# Autodesk Inventor assembly: Тиски
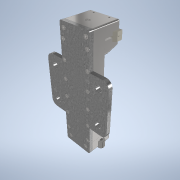
[picture p0: Inventor's stored thumbnail of the model, 180x180]
Saved by Autodesk Inventor 2020 (Build 240168000, 168)
## iProperties
Created: 2020-12-05
Part Number: Тиски
Document SubType Name: Assembly
Designer: User
Author: User
## Documents named in this file (18)
- F:\Детали\Тиски\Тиски.iam
- F:\Детали\Тиски\Основание.ipt
- F:\Детали\Тиски\Тиски\Мастер проектирования\Болтовое соединение1.iam
- F:\Детали\Тиски\Упор 1.ipt
- F:\Детали\Тиски\Упор 2.ipt
- F:\Детали\Тиски\Направляющая.ipt
- F:\Детали\Тиски\Тиски\Мастер проектирования\Болтовое соединение3.iam
- F:\Детали\Тиски\Губка.ipt
- F:\Детали\Тиски\Тиски\Мастер проектирования\Болтовое соединение5.iam
- F:\Детали\Тиски\Каретка.ipt
- F:\Детали\Тиски\Тиски\Мастер проектирования\Подшипник1.iam
- F:\Детали\Тиски\Вал1.ipt
- F:\Детали\Тиски\Фланец.ipt
- C:\Users\User\Documents\Inventor\Content Center Files\R2020\ru-RU\DIN 916\DIN 916 - M4  x  10.ipt
- F:\Детали\Тиски\Тиски\Мастер проектирования\Болтовое соединение7.iam
- F:\Детали\Тиски\Привод.iam
- F:\Детали\Тиски\Тиски\Мастер проектирования\Болтовое соединение8.iam
- F:\Детали\Тиски\Ручка.ipt
## Components (21 placed, 13 different names)
1. Основание:1 — Заподлицо:1, Совмещение:4, Совмещение:5, Совмещение:6, Совмещение:7, Совмещение:8, Совмещение:9, Совмещение:10, Совмещение:11, Совмещение:12, Совмещение:13, Совмещение:14, Совмещение:15, Совмещение:17, Совмещение:19, Совмещение:21, Совмещение:23, Совмещение:25, Совмещение:27, Совмещение:29, Совмещение:31, Совмещение:33, Совмещение:35, Совмещение:40, Совмещение:41, Совмещение:42, Совмещение:43, Совмещение:44, Совмещение:46, Совмещение:48, Совмещение:50, Совмещение:57, Совмещение:59, Совмещение:61, Жесткий:1, Жесткий:2, Жесткий:3, Совмещение:82, Совмещение:83, Совмещение:93
2. Болтовое соединение:1 [sub-assembly] — Совмещение:59, Совмещение:60, Совмещение:61
3. Упор 1:1 — Жесткий:2, Жесткий:4, С поворотом:2
4. Упор 2:1 — Жесткий:3, С поворотом:1
5. Направляющая:1 — Жесткий:1, Совмещение:81, Угол:1
6. Болтовое соединение:2 [sub-assembly] — Совмещение:93, Совмещение:94
7. Губка:1 — Жесткий:4, Совмещение:70, Совмещение:71, Совмещение:72, Совмещение:74, Совмещение:76
8. Болтовое соединение:3 [sub-assembly] — Совмещение:76, Совмещение:77
9. Каретка:1 — Совмещение:80, Совмещение:81, ЗубчПер:1, Жесткий:8
10. Подшипник:1 [sub-assembly] — С поворотом:1
11. Подшипник:2 [sub-assembly] — С поворотом:2, Совмещение:92
12. Вал:1 — Жесткий:5, Совмещение:80, ЗубчПер:1, Совмещение:92, Угол:1
13. Фланец:1 — Жесткий:5, Жесткий:6, Жесткий:7
14. DIN 916 M4  x  10:1 — Жесткий:6
15. DIN 916 M4  x  10:2 — Жесткий:7
16. Губка:2 — Жесткий:8, Совмещение:84, Совмещение:85, Совмещение:86, Совмещение:88, Совмещение:90
17. Болтовое соединение:4 [sub-assembly] — Совмещение:90, Совмещение:91
18. Привод:1 [sub-assembly] — Совмещение:95, Совмещение:96, С поворотом:3
19. Болтовое соединение:5 [sub-assembly] — Совмещение:95, Совмещение:96, Заподлицо:2
20. Ручка:1 — Заподлицо:2
21. Ручка:2 — С поворотом:3
## Relationships (90: Mate 75, WeldJoint 8, RevoluteJoint 3, Flush 2, RelateRotation 1, Angle 1)
- Заподлицо:1 [Flush] (-3.3 mm): Основание:1
- Совмещение:4 [Mate]: Основание:1
- Совмещение:5 [Mate]: Основание:1
- Совмещение:6 [Mate]: Основание:1
- Совмещение:7 [Mate]: Основание:1
- Совмещение:8 [Mate]: Основание:1
- Совмещение:9 [Mate]: Основание:1
- Совмещение:10 [Mate]: Основание:1
- Совмещение:11 [Mate]: Основание:1
- Совмещение:12 [Mate]: Основание:1
- Совмещение:13 [Mate]: Основание:1
- Совмещение:14 [Mate]: Основание:1
- Совмещение:15 [Mate]: Основание:1
- Совмещение:16 [Mate]
- Совмещение:17 [Mate]: Основание:1
- Совмещение:18 [Mate]
- Совмещение:19 [Mate]: Основание:1
- Совмещение:20 [Mate]
- Совмещение:21 [Mate]: Основание:1
- Совмещение:22 [Mate]
- Совмещение:23 [Mate]: Основание:1
- Совмещение:24 [Mate]
- Совмещение:25 [Mate]: Основание:1
- Совмещение:26 [Mate]
- Совмещение:27 [Mate]: Основание:1
- Совмещение:28 [Mate]
- Совмещение:29 [Mate]: Основание:1
- Совмещение:30 [Mate]
- Совмещение:31 [Mate]: Основание:1
- Совмещение:32 [Mate]
- Совмещение:33 [Mate]: Основание:1
- Совмещение:34 [Mate]
- Совмещение:35 [Mate]: Основание:1
- Совмещение:36 [Mate]
- Совмещение:40 [Mate]: Основание:1
- Совмещение:41 [Mate]: Основание:1
- Совмещение:42 [Mate]: Основание:1
- Совмещение:43 [Mate]: Основание:1
- Совмещение:44 [Mate]: Основание:1
- Совмещение:45 [Mate]
- Совмещение:46 [Mate]: Основание:1
- Совмещение:47 [Mate]
- Совмещение:48 [Mate]: Основание:1
- Совмещение:49 [Mate]
- Совмещение:50 [Mate]: Основание:1
- Совмещение:51 [Mate]
- Совмещение:57 [Mate]: Основание:1
- Совмещение:58 [Mate]
- Совмещение:59 [Mate]: Основание:1 ↔ Болтовое соединение:1
- Совмещение:60 [Mate]: Болтовое соединение:1
- Совмещение:61 [Mate]: Основание:1 ↔ Болтовое соединение:1
- Жесткий:1 [WeldJoint] (-30 mm): Основание:1 ↔ Направляющая:1
- Жесткий:2 [WeldJoint]: Основание:1 ↔ Упор 1:1
- Жесткий:3 [WeldJoint]: Основание:1 ↔ Упор 2:1
- Жесткий:4 [WeldJoint]: Упор 1:1 ↔ Губка:1
- Совмещение:70 [Mate]: Губка:1
- Совмещение:71 [Mate]: Губка:1
- Совмещение:72 [Mate]: Губка:1
- Совмещение:73 [Mate]
- Совмещение:74 [Mate]: Губка:1
- Совмещение:75 [Mate]
- Совмещение:76 [Mate]: Губка:1 ↔ Болтовое соединение:3
- Совмещение:77 [Mate]: Болтовое соединение:3
- С поворотом:1 [RevoluteJoint]: Упор 2:1 ↔ Подшипник:1
- С поворотом:2 [RevoluteJoint]: Упор 1:1 ↔ Подшипник:2
- Жесткий:5 [WeldJoint] (-16 mm): Вал:1 ↔ Фланец:1
- Совмещение:80 [Mate]: Каретка:1 ↔ Вал:1
- Совмещение:81 [Mate]: Направляющая:1 ↔ Каретка:1
- ЗубчПер:1 [RelateRotation] (1.032 ul): Каретка:1 ↔ Вал:1
- Совмещение:82 [Mate]: Основание:1
- Совмещение:83 [Mate]: Основание:1
- Жесткий:6 [WeldJoint] (-1 mm): Фланец:1 ↔ DIN 916 M4  x  10:1
- Жесткий:7 [WeldJoint] (-1 mm): Фланец:1 ↔ DIN 916 M4  x  10:2
- Жесткий:8 [WeldJoint]: Каретка:1 ↔ Губка:2
- Совмещение:84 [Mate]: Губка:2
- Совмещение:85 [Mate]: Губка:2
- Совмещение:86 [Mate]: Губка:2
- Совмещение:87 [Mate]
- Совмещение:88 [Mate]: Губка:2
- Совмещение:89 [Mate]
- Совмещение:90 [Mate]: Губка:2 ↔ Болтовое соединение:4
- Совмещение:91 [Mate]: Болтовое соединение:4
- Совмещение:92 [Mate]: Подшипник:2 ↔ Вал:1
- Угол:1 [Angle] (0 deg): Направляющая:1 ↔ Вал:1
- Совмещение:93 [Mate]: Основание:1 ↔ Болтовое соединение:2
- Совмещение:94 [Mate]: Болтовое соединение:2
- Совмещение:95 [Mate]: Привод:1 ↔ Болтовое соединение:5
- Совмещение:96 [Mate]: Привод:1 ↔ Болтовое соединение:5
- Заподлицо:2 [Flush]: Болтовое соединение:5 ↔ Ручка:1
- С поворотом:3 [RevoluteJoint]: Привод:1 ↔ Ручка:2
